# Autodesk Inventor assembly: ladder
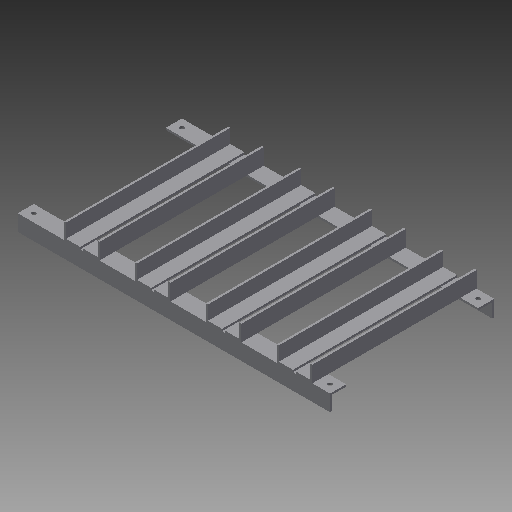
[picture p0: Inventor's stored thumbnail of the model, 512x512]
Saved by Autodesk Inventor 2017 (Build 210142000, 142)
## iProperties
Created: 2018-10-22
Part Number: ladder
Document SubType Name: Assembly
Designer: ddeboer
Author: ddeboer
Title: Ladder
## Documents named in this file (3)
- C:\Users\ddeboer\Desktop\snap_holder\ladder.iam
- C:\Users\ddeboer\Desktop\snap_holder\angle_L1.ipt
- C:\Users\ddeboer\Desktop\snap_holder\angle_M.ipt
## Components (10 placed, 3 different names)
1. angle_L1:front — Flush:1, Mate:1, Flush:2, Flush:3, Mate:2, Flush:4, Mate:3, Flush:5
2. angle_L1:back — Flush:1, Mate:1, Flush:2
3. angle_M:1 — Flush:3, Mate:2, Flush:4, Mate:4
4. angle_M:2 — Mate:3, Flush:5, Mate:4
5. angle_M:3
6. angle_M:4
7. angle_M:5
8. angle_M:6
9. angle_M:7
10. angle_M:8
## Component patterns: (4 elements, first: angle_M:1 + angle_M:2)
## Relationships (9: Flush 5, Mate 4)
- Flush:1: angle_L1:front ↔ angle_L1:back
- Mate:1 (252.4252 mm): angle_L1:front ↔ angle_L1:back
- Flush:2: angle_L1:front ↔ angle_L1:back
- Flush:3: angle_L1:front ↔ angle_M:1
- Mate:2: angle_L1:front ↔ angle_M:1
- Flush:4 (73.025 mm): angle_L1:front ↔ angle_M:1
- Mate:3: angle_L1:front ↔ angle_M:2
- Flush:5: angle_L1:front ↔ angle_M:2
- Mate:4 (49.53 mm): angle_M:1 ↔ angle_M:2
